# Autodesk Inventor assembly: 5 Barras Version 0
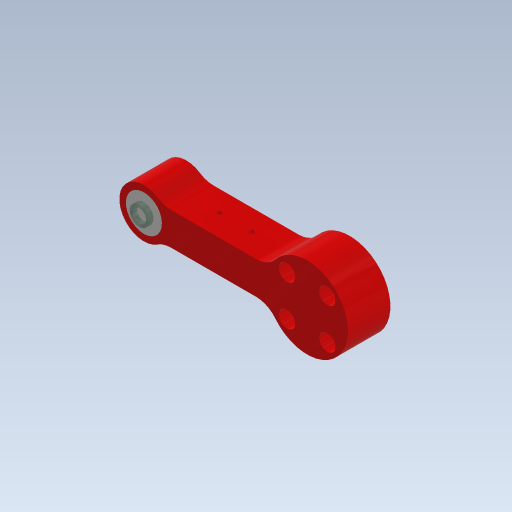
[picture p0: Inventor's stored thumbnail of the model, 512x512]
Saved by Autodesk Inventor 2024.2 (Build 282272000, 272)
## iProperties
Created: 2025-02-06
Part Number: 5 Barras Version 0
Document SubType Name: Assembly
Designer: jp.reyesf
Mass: 187.02 g
Surface Area: 264.613 cm^2
Volume: 97.4899 cm^3
Density: 1.91835 g/cm^3
Author: jp.reyesf
## Documents named in this file (7)
- C:\Users\jp.reyesf\Desktop\Master-Thesis\five_bar\assets\CAD\Robot\Subassemblies\Proximal Link 2.iam
- C:\Users\jp.reyesf\Desktop\Master-Thesis\five_bar\assets\CAD\Robot\Proximal Link 1.ipt
- C:\Users\jp.reyesf\Desktop\Master-Thesis\five_bar\assets\CAD\Robot\Spacer.ipt
- C:\Users\jp.reyesf\Desktop\Master-Thesis\five_bar\assets\CAD\Robot\Bearing.ipt
- C:\Users\jp.reyesf\Desktop\Master-Thesis\five_bar\assets\CAD\Robot\separator.ipt
- C:\Users\jp.reyesf\Desktop\Master-Thesis\five_bar\assets\CAD\Robot\rod.ipt
- C:\Users\jp.reyesf\Desktop\Master-Thesis\five_bar\assets\CAD\Robot\Subassemblies\DummyBar.ipt
## Components (7 placed, 6 different names)
1. Proximal Link 1:1 — Mate:30, Flush:1, Mate:37, Mate:52, Flush:2, Mate:53, Flush:3, Angle:1, Mate:54, Mate:55, Flush:4
2. separator:1 — Mate:37, Mate:54
3. Spacer:4 — Mate:30
4. Bearing:8 — Flush:1
5. Bearing:9
6. rod:1 — Mate:52, Flush:2
7. DummyBar:1 — Mate:55, Flush:4
## Relationships (15: Mate 10, Flush 4, Angle 1)
- [Mate]: Spacer:4 ↔ Bearing:8
- [Mate]: Spacer:4 ↔ Bearing:9
- [Mate]: Spacer:4 ↔ Bearing:8
- [Mate]: Spacer:4 ↔ Bearing:9
- Mate:30: Proximal Link 1:1 ↔ Spacer:4
- Flush:1: Proximal Link 1:1 ↔ Bearing:8
- Mate:37: Proximal Link 1:1 ↔ separator:1
- Mate:52: Proximal Link 1:1 ↔ rod:1
- Flush:2: Proximal Link 1:1 ↔ rod:1
- Mate:53: Proximal Link 1:1
- Flush:3: Proximal Link 1:1
- Angle:1 (0 deg): Proximal Link 1:1
- Mate:54: Proximal Link 1:1 ↔ separator:1
- Mate:55: Proximal Link 1:1 ↔ DummyBar:1
- Flush:4: Proximal Link 1:1 ↔ DummyBar:1
## Named parameters: d26_d14 = 0 mm, d27_d15 = 0 mm, d28_d16 = 0 mm, d29_d17 = 0 mm
